# Autodesk Inventor assembly: ЛЦМК0000002.00.00.00.00.10
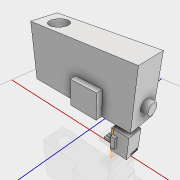
[picture p0: Inventor's stored thumbnail of the model, 180x180]
Saved by Autodesk Inventor 2021.2 (Build 252289000, 289)
## iProperties
Created: 2025-10-23
Part Number: ЛЦМК0000002.00.00.00.00.10
Document SubType Name: Assembly
Designer: Захаров
Author: Захаров
## Documents named in this file (3)
- C:\Users\User\Documents\ARHeadGen1\ЛЦМК0000002.00.00.00.00.10.iam
- C:\Users\User\Documents\ARHeadGen1\ЛЦМК0000002.00.00.00.00.05.ipt
- C:\Users\User\Documents\ARHeadGen1\Сборка1.iam
## Components (2 placed, 2 different names)
1. ЛЦМК0000002.00.00.00.00.05:1 — Совмещение:1, Заподлицо:1, Заподлицо:2
2. Сборка1:1 [sub-assembly] — Совмещение:1, Заподлицо:1, Заподлицо:2
## Relationships (3: Flush 2, Mate 1)
- Совмещение:1 [Mate] (3 mm): ЛЦМК0000002.00.00.00.00.05:1 ↔ Сборка1:1
- Заподлицо:1 [Flush]: ЛЦМК0000002.00.00.00.00.05:1 ↔ Сборка1:1
- Заподлицо:2 [Flush] (3 mm): ЛЦМК0000002.00.00.00.00.05:1 ↔ Сборка1:1
